# Autodesk Inventor assembly: rollerassembly(v3)
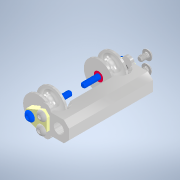
[picture p0: Inventor's stored thumbnail of the model, 180x180]
Saved by Autodesk Inventor 2022 (Build 260153000, 153)
## iProperties
Created: 2022-11-15
Part Number: rollerassembly(v3)
Document SubType Name: Assembly
Designer: matia
Author: matia
## Documents named in this file (7)
- C:\Users\matia\Desktop\1QuadMod\rollers\rollerassembly(v3).iam
- C:\Users\matia\Desktop\1QuadMod\rollerbase(v2).ipt
- C:\Users\matia\Desktop\1QuadMod\rollertriangle(v3).ipt
- C:\Users\matia\Desktop\1QuadMod\screws\92949A330_18-8 Stainless Steel Button Head Hex Drive Screw.ipt
- C:\Users\matia\Desktop\1QuadMod\wheel.ipt
- C:\Users\matia\Desktop\1QuadMod\wheelbushing.ipt
- C:\Users\matia\Desktop\1QuadMod\screws\92949A333_18-8 Stainless Steel Button Head Hex Drive Screw.ipt
## Components (13 placed, 6 different names)
1. rollerbase(v2):1 — Mate:1, Mate:2, Mate:3, Mate:4, Mate:17
2. rollertriangle(v3):1 — Mate:3, Mate:4, Mate:7, Mate:8, Mate:14, Mate:17
3. rollertriangle(v3):2 — Mate:1, Mate:2, Mate:5, Mate:6, Mate:13
4. 92949A330_18-8 Stainless Steel Button Head Hex Drive Screw:1 — Mate:6
5. 92949A330_18-8 Stainless Steel Button Head Hex Drive Screw:2 — Mate:5
6. 92949A330_18-8 Stainless Steel Button Head Hex Drive Screw:3 — Mate:8
7. 92949A330_18-8 Stainless Steel Button Head Hex Drive Screw:4 — Mate:7
8. wheel:1 — Mate:9, Mate:10
9. wheel:2 — Mate:11, Mate:12
10. wheelbushing:1 — Mate:9, Mate:10, Mate:15
11. wheelbushing:2 — Mate:11, Mate:12, Mate:16
12. 92949A333_18-8 Stainless Steel Button Head Hex Drive Screw:1 — Mate:13, Mate:15
13. 92949A333_18-8 Stainless Steel Button Head Hex Drive Screw:2 — Mate:14, Mate:16
## Relationships (17: Mate 17)
- Mate:1: rollerbase(v2):1 ↔ rollertriangle(v3):2
- Mate:2: rollerbase(v2):1 ↔ rollertriangle(v3):2
- Mate:3: rollerbase(v2):1 ↔ rollertriangle(v3):1
- Mate:4: rollerbase(v2):1 ↔ rollertriangle(v3):1
- Mate:5: rollertriangle(v3):2 ↔ 92949A330_18-8 Stainless Steel Button Head Hex Drive Screw:2
- Mate:6: rollertriangle(v3):2 ↔ 92949A330_18-8 Stainless Steel Button Head Hex Drive Screw:1
- Mate:7: rollertriangle(v3):1 ↔ 92949A330_18-8 Stainless Steel Button Head Hex Drive Screw:4
- Mate:8: rollertriangle(v3):1 ↔ 92949A330_18-8 Stainless Steel Button Head Hex Drive Screw:3
- Mate:9: wheel:1 ↔ wheelbushing:1
- Mate:10: wheel:1 ↔ wheelbushing:1
- Mate:11: wheel:2 ↔ wheelbushing:2
- Mate:12: wheel:2 ↔ wheelbushing:2
- Mate:13: rollertriangle(v3):2 ↔ 92949A333_18-8 Stainless Steel Button Head Hex Drive Screw:1
- Mate:14: rollertriangle(v3):1 ↔ 92949A333_18-8 Stainless Steel Button Head Hex Drive Screw:2
- Mate:15: wheelbushing:1 ↔ 92949A333_18-8 Stainless Steel Button Head Hex Drive Screw:1
- Mate:16: wheelbushing:2 ↔ 92949A333_18-8 Stainless Steel Button Head Hex Drive Screw:2
- Mate:17: rollerbase(v2):1 ↔ rollertriangle(v3):1
